# Autodesk Inventor assembly: remmy
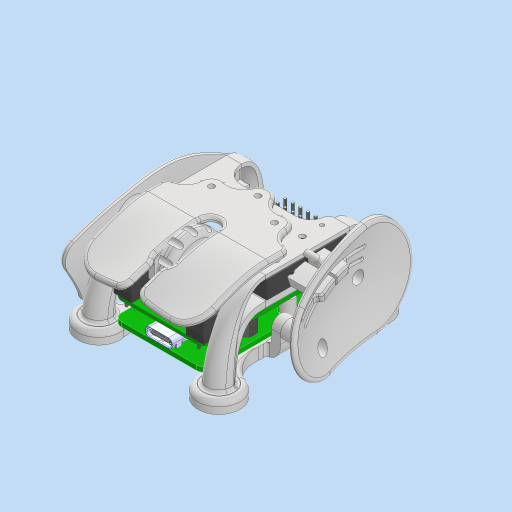
[picture p0: Inventor's stored thumbnail of the model, 512x512]
Saved by Autodesk Inventor 2024 (Build 280153000, 153)
## iProperties
Created: 2025-05-08
Part Number: remmy
Document SubType Name: Assembly
Designer: XxPan
Author: XxPan
## Documents named in this file (9)
- D:\The Mind Palace\remmy_mouse\CAD\remmy.iam
- D:\The Mind Palace\remmy_mouse\CAD\mcu_board.iam
- D:\The Mind Palace\remmy_mouse\CAD\sensor_board.iam
- D:\The Mind Palace\remmy_mouse\CAD\M3_H8.0mm_board_spacer.ipt
- D:\The Mind Palace\remmy_mouse\CAD\shell\mouse_buttons_1-2.ipt
- D:\The Mind Palace\remmy_mouse\CAD\shell\thumb_pad_shortened.ipt
- D:\The Mind Palace\remmy_mouse\CAD\shell\pinky_pad_v2.ipt
- D:\The Mind Palace\remmy_mouse\CAD\shell\base_plate.ipt
- D:\The Mind Palace\remmy_mouse\CAD\socket_head_cap_screw_M3x5.ipt
## Components (16 placed, 8 different names)
1. mcu_board:1 [sub-assembly] — Insert:5, Insert:6, Insert:7, Insert:8
2. sensor_board:1 [sub-assembly] — Flush:1, Flush:2, Flush:3, Insert:1, Insert:2, Insert:3, Insert:4, Mate:1
3. thumb_pad_shortened:1 — Mate:2, Flush:7
4. pinky_pad_v2:1 — Flush:8, Mate:3
5. mouse_buttons_1-2:1 — Mate:4, Insert:13, Insert:14
6. M3_H8.0mm_board_spacer:1 — Insert:1
7. M3_H8.0mm_board_spacer:2 — Insert:3, Insert:5
8. M3_H8.0mm_board_spacer:3 — Insert:2, Insert:6
9. M3_H8.0mm_board_spacer:4 — Insert:4
10. base_plate:1 — Flush:4, Flush:6, Mate:1, Insert:9, Insert:10, Insert:11, Insert:12, Mate:2, Flush:7, Flush:8, Mate:3, Mate:4, Insert:13, Insert:14
11. socket_head_cap_screw_M3x5:1 — Insert:7
12. socket_head_cap_screw_M3x5:2 — Insert:8
13. socket_head_cap_screw_M3x5:3 — Insert:10
14. socket_head_cap_screw_M3x5:4 — Insert:9
15. socket_head_cap_screw_M3x5:5 — Insert:12
16. socket_head_cap_screw_M3x5:6 — Insert:11
## Relationships (25: Insert 14, Flush 7, Mate 4)
- Flush:1: sensor_board:1
- Flush:2: sensor_board:1
- Flush:3: sensor_board:1
- Insert:1: sensor_board:1 ↔ M3_H8.0mm_board_spacer:1
- Insert:2: sensor_board:1 ↔ M3_H8.0mm_board_spacer:3
- Insert:3: sensor_board:1 ↔ M3_H8.0mm_board_spacer:2
- Insert:4: sensor_board:1 ↔ M3_H8.0mm_board_spacer:4
- Insert:5: mcu_board:1 ↔ M3_H8.0mm_board_spacer:2
- Insert:6: mcu_board:1 ↔ M3_H8.0mm_board_spacer:3
- Flush:4: base_plate:1
- Flush:6: base_plate:1
- Mate:1: sensor_board:1 ↔ base_plate:1
- Insert:7: mcu_board:1 ↔ socket_head_cap_screw_M3x5:1
- Insert:8: mcu_board:1 ↔ socket_head_cap_screw_M3x5:2
- Insert:9: base_plate:1 ↔ socket_head_cap_screw_M3x5:4
- Insert:10: base_plate:1 ↔ socket_head_cap_screw_M3x5:3
- Insert:11: base_plate:1 ↔ socket_head_cap_screw_M3x5:6
- Insert:12: base_plate:1 ↔ socket_head_cap_screw_M3x5:5
- Mate:2: thumb_pad_shortened:1 ↔ base_plate:1
- Flush:7 (2 mm): thumb_pad_shortened:1 ↔ base_plate:1
- Flush:8 (2 mm): pinky_pad_v2:1 ↔ base_plate:1
- Mate:3: pinky_pad_v2:1 ↔ base_plate:1
- Mate:4: mouse_buttons_1-2:1 ↔ base_plate:1
- Insert:13: mouse_buttons_1-2:1 ↔ base_plate:1
- Insert:14: mouse_buttons_1-2:1 ↔ base_plate:1
